# Autodesk Inventor assembly: 2018 Scissor R
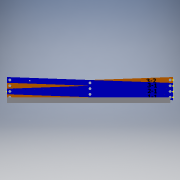
[picture p0: Inventor's stored thumbnail of the model, 180x180]
Saved by Autodesk Inventor 2018 (Build 220112000, 112)
## iProperties
Created: 2018-01-28
Part Number: 2018 Scissor R
Document SubType Name: Assembly
Designer: Apple
Author: Apple
## Documents named in this file (8)
- C:\Users\Apple\Documents\Inventor\2018 PowerUp\2018 Scissor\2018 Scissor R.iam
- C:\Users\Apple\Documents\Inventor\2018 PowerUp\2018 Scissor\2018 Slide.ipt
- C:\Users\Apple\Documents\Inventor\2018 PowerUp\2018 Scissor\2018 Bar1_1.ipt
- C:\Users\Apple\Documents\Inventor\2018 PowerUp\2018 Scissor\2018 Bar1_2.ipt
- C:\Users\Apple\Documents\Inventor\2018 PowerUp\2018 Scissor\2018 Bar2_1.ipt
- C:\Users\Apple\Documents\Inventor\2018 PowerUp\2018 Scissor\2018 Bar2_2.ipt
- C:\Users\Apple\Documents\Inventor\2018 PowerUp\2018 Scissor\2018 Bar3_1.ipt
- C:\Users\Apple\Documents\Inventor\2018 PowerUp\2018 Scissor\2018 Bar3_2.ipt
## Components (7 placed, 7 different names)
1. 2018 Slide:1 — Mate:1, Mate:2, Mate:17
2. 2018 Bar1_2:1 — Mate:1, Mate:2, Mate:3, Mate:6, Mate:7, Mate:10, Mate:12
3. 2018 Bar1_1:1 — Angle:1, Mate:3, Mate:6, Mate:7, Mate:11, Mate:17
4. 2018 Bar2_1:1 — Angle:2, Mate:4, Mate:8, Mate:9, Mate:10, Mate:12, Mate:16
5. 2018 Bar2_2:1 — Angle:1, Mate:4, Mate:8, Mate:9, Mate:11, Mate:15
6. 2018 Bar3_1:1 — Mate:5, Mate:13, Mate:14, Mate:15
7. 2018 Bar3_2:1 — Angle:2, Mate:5, Mate:13, Mate:14, Mate:16
## Relationships (19: Mate 17, Angle 2)
- Mate:1: 2018 Slide:1 ↔ 2018 Bar1_2:1
- Mate:2: 2018 Slide:1 ↔ 2018 Bar1_2:1
- Angle:1 (4.1 deg): 2018 Bar1_1:1 ↔ 2018 Bar2_2:1
- Angle:2 (4.1 deg): 2018 Bar2_1:1 ↔ 2018 Bar3_2:1
- Mate:3: 2018 Bar1_2:1 ↔ 2018 Bar1_1:1
- Mate:4: 2018 Bar2_1:1 ↔ 2018 Bar2_2:1
- Mate:5: 2018 Bar3_1:1 ↔ 2018 Bar3_2:1
- Mate:6: 2018 Bar1_2:1 ↔ 2018 Bar1_1:1
- Mate:7: 2018 Bar1_2:1 ↔ 2018 Bar1_1:1
- Mate:8: 2018 Bar2_1:1 ↔ 2018 Bar2_2:1
- Mate:9: 2018 Bar2_1:1 ↔ 2018 Bar2_2:1
- Mate:10: 2018 Bar1_2:1 ↔ 2018 Bar2_1:1
- Mate:11: 2018 Bar1_1:1 ↔ 2018 Bar2_2:1
- Mate:12: 2018 Bar1_2:1 ↔ 2018 Bar2_1:1
- Mate:13: 2018 Bar3_1:1 ↔ 2018 Bar3_2:1
- Mate:14: 2018 Bar3_1:1 ↔ 2018 Bar3_2:1
- Mate:15: 2018 Bar2_2:1 ↔ 2018 Bar3_1:1
- Mate:16: 2018 Bar2_1:1 ↔ 2018 Bar3_2:1
- Mate:17: 2018 Slide:1 ↔ 2018 Bar1_1:1
